# Autodesk Inventor assembly: distancias
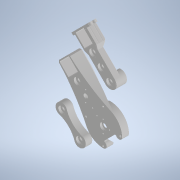
[picture p0: Inventor's stored thumbnail of the model, 180x180]
Saved by Autodesk Inventor 2021 (Build 250183000, 183)
## iProperties
Created: 2021-04-04
Part Number: distancias
Document SubType Name: Assembly
Designer: jorge
Author: jorge
## Documents named in this file (4)
- D:\Documentos\Inventor\Telescopio\distancias.iam
- D:\Documentos\Inventor\Telescopio\Union_fija_lazy_susan_2_1.ipt
- D:\Documentos\Inventor\Telescopio\Reduccion_Theta_3_reducciones_1.ipt
- D:\Documentos\Inventor\Telescopio\Distancia_Cojinetes_2.ipt
## Components (3 placed, 3 different names)
1. Union_fija_lazy_susan_2_1:1 — Mate:1, Mate:2, Mate:3, Mate:4
2. Reduccion_Theta_3_reducciones_1:1 — Mate:1, Mate:2
3. Distancia_Cojinetes_2:1 — Mate:3, Mate:4
## Relationships (4: Mate 4)
- Mate:1: Union_fija_lazy_susan_2_1:1 ↔ Reduccion_Theta_3_reducciones_1:1
- Mate:2: Union_fija_lazy_susan_2_1:1 ↔ Reduccion_Theta_3_reducciones_1:1
- Mate:3: Union_fija_lazy_susan_2_1:1 ↔ Distancia_Cojinetes_2:1
- Mate:4: Union_fija_lazy_susan_2_1:1 ↔ Distancia_Cojinetes_2:1
